# Autodesk Inventor assembly: converter
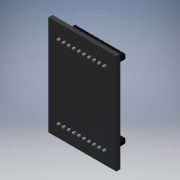
[picture p0: Inventor's stored thumbnail of the model, 180x180]
Saved by Autodesk Inventor 2016 (Build 200138000, 138)
## iProperties
Created: 2016-10-13
Part Number: converter
Document SubType Name: Assembly
Designer: Jakub
Author: Jakub
## Documents named in this file (3)
- C:\Users\Jakub\Documents\DATA BANK\Projekty\Dron\Enix\V3\kamamiLogicVoltageConverter\converter.iam
- C:\Users\Jakub\Documents\DATA BANK\Projekty\Dron\Enix\V3\kamamiLogicVoltageConverter\pcb.ipt
- C:\Users\Jakub\Documents\DATA BANK\Projekty\Dron\Enix\V3\kamamiLogicVoltageConverter\Header5.ipt
## Components (5 placed, 2 different names)
1. pcb:1 — Mate:1, Mate:2, Mate:3, Mate:4, Mate:5, Mate:6, Mate:7, Mate:8
2. Header5:1 — Mate:1, Mate:3
3. Header5:2 — Mate:2, Mate:4
4. Header5:3 — Mate:6, Mate:8
5. Header5:4 — Mate:5, Mate:7
## Relationships (8: Mate 8)
- Mate:1: pcb:1 ↔ Header5:1
- Mate:2: pcb:1 ↔ Header5:2
- Mate:3: pcb:1 ↔ Header5:1
- Mate:4: pcb:1 ↔ Header5:2
- Mate:5: pcb:1 ↔ Header5:4
- Mate:6: pcb:1 ↔ Header5:3
- Mate:7: pcb:1 ↔ Header5:4
- Mate:8: pcb:1 ↔ Header5:3
